# Autodesk Inventor assembly: 2016 plate with 2018 boxes
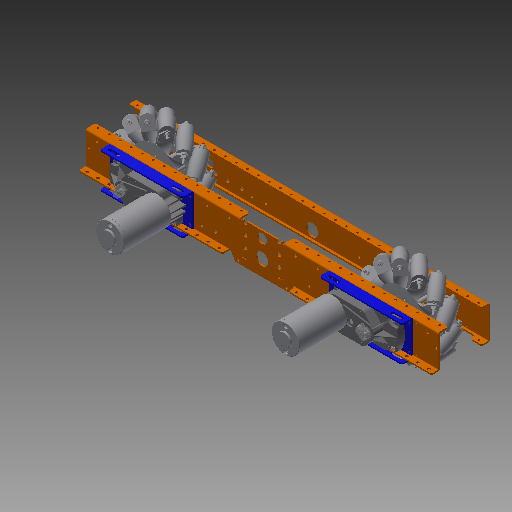
[picture p0: Inventor's stored thumbnail of the model, 512x512]
Saved by Autodesk Inventor 2018 (Build 220112000, 112)
## iProperties
Created: 2018-01-16
Part Number: 2016 plate with 2018 boxes
Document SubType Name: Assembly
Designer: Apple
Author: Apple
## Documents named in this file (8)
- C:\Users\Apple\Documents\Inventor\2018 PowerUp\2016 plate with 2018 boxes.iam
- C:\Users\Apple\Documents\Inventor\2018 PowerUp\2018 am-2952 AM14U2 Inside Sheet.ipt.ipt
- C:\Users\Apple\Documents\Inventor\2018 PowerUp\2016_Files_2018_Mod\Assembly\Imported Components\8-mecanum-right-with-roller\8-mecanum-right-with-roller.iam
- C:\Users\Apple\Documents\Inventor\2018 PowerUp\2018 am-2951 AM14U2 Outside Sheet.ipt.ipt
- C:\Users\Apple\Documents\Inventor\2018 PowerUp\2018ToughboxMicrowithAngledPlateAndCim.iam
- C:\Users\Apple\Documents\Inventor\2018 PowerUp\AndyMark\15-697867_CAD files\15-697867_CAD files\final.ipt
- 2018 am-2952 AM14U2 Inside Sheet.ipt
- 2018 am-2951 AM14U2 Outside Sheet.ipt
## Components (8 placed, 5 different names)
1. 2018 am-2952 AM14U2 Inside Sheet.ipt:1 — Mate:7, Flush:2, Flush:3, Flush:6, Mate:8, Mate:9, Mate:10, Mate:11
2. 8-mecanum-right-with-roller:2 [sub-assembly] — Flush:5, Flush:6
3. 8-mecanum-right-with-roller:3 [sub-assembly] — Flush:5
4. 2018 am-2951 AM14U2 Outside Sheet.ipt:1 — Mate:7, Flush:2, Flush:3
5. 2018ToughboxMicrowithAngledPlateAndCim:1 [sub-assembly] — Mate:9, Mate:10, Flush:7, Mate:22, Mate:23
6. 2018ToughboxMicrowithAngledPlateAndCim:2 [sub-assembly] — Mate:8, Mate:11, Flush:7, Mate:20, Mate:21
7. final:1 — Mate:20, Mate:21
8. final:2 — Mate:22, Mate:23
## Relationships (14: Mate 9, Flush 5)
- Mate:7 (112.3442 mm): 2018 am-2952 AM14U2 Inside Sheet.ipt:1 ↔ 2018 am-2951 AM14U2 Outside Sheet.ipt:1
- Flush:2: 2018 am-2952 AM14U2 Inside Sheet.ipt:1 ↔ 2018 am-2951 AM14U2 Outside Sheet.ipt:1
- Flush:3: 2018 am-2952 AM14U2 Inside Sheet.ipt:1 ↔ 2018 am-2951 AM14U2 Outside Sheet.ipt:1
- Flush:5: 8-mecanum-right-with-roller:2 ↔ 8-mecanum-right-with-roller:3
- Flush:6 (-80 mm): 2018 am-2952 AM14U2 Inside Sheet.ipt:1 ↔ 8-mecanum-right-with-roller:2
- Mate:8: 2018 am-2952 AM14U2 Inside Sheet.ipt:1 ↔ 2018ToughboxMicrowithAngledPlateAndCim:2
- Mate:9: 2018 am-2952 AM14U2 Inside Sheet.ipt:1 ↔ 2018ToughboxMicrowithAngledPlateAndCim:1
- Mate:10: 2018 am-2952 AM14U2 Inside Sheet.ipt:1 ↔ 2018ToughboxMicrowithAngledPlateAndCim:1
- Mate:11: 2018 am-2952 AM14U2 Inside Sheet.ipt:1 ↔ 2018ToughboxMicrowithAngledPlateAndCim:2
- Flush:7: 2018ToughboxMicrowithAngledPlateAndCim:1 ↔ 2018ToughboxMicrowithAngledPlateAndCim:2
- Mate:20: 2018ToughboxMicrowithAngledPlateAndCim:2 ↔ final:1
- Mate:21: 2018ToughboxMicrowithAngledPlateAndCim:2 ↔ final:1
- Mate:22: 2018ToughboxMicrowithAngledPlateAndCim:1 ↔ final:2
- Mate:23: 2018ToughboxMicrowithAngledPlateAndCim:1 ↔ final:2
